# Autodesk Inventor assembly: buck-converter-din-rail-mount
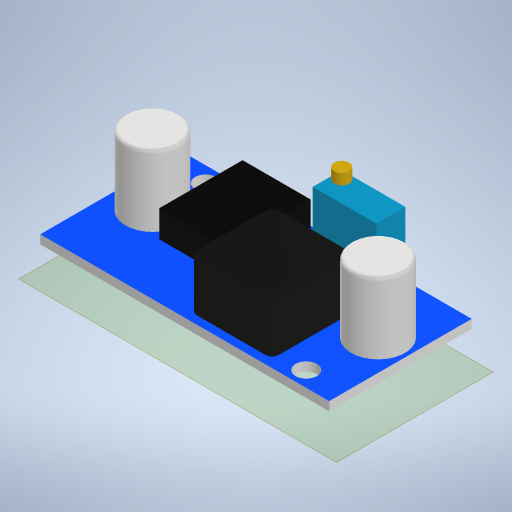
[picture p0: Inventor's stored thumbnail of the model, 512x512]
Saved by Autodesk Inventor 2023 (Build 270158030, 158C)
## iProperties
Created: 2024-03-29
Part Number: buck-converter-din-rail-mount
Document SubType Name: Assembly
Designer: Imogen Heard
Author: Imogen Heard
## iProperties of the stored document Power Buck Converter.ipt
Created: 2022-05-13
Part Number: Power Buck Converter
Material: Generic
Document SubType Name: Modeling
Designer: Imogen Heard
Density: 1 g/cm^3
Appearance: Default
Title: D:\Inventor\STEP FOR KICAD\Power Buck Converter.stp
Author: dech3
Sending System: Autodesk Inventor 2022
Preprocessor: ST-DEVELOPER v18.1
## Documents named in this file (3)
- **C:\Users\dheard\Documents\0004-inventor\Inventor_Projects\electronics-enclosure\buck-converter-din-rail-mount.iam*LocalDocs*xAaaaqqcaAaaaaaaaAaaaqi10Rg*Power Buck Converter.ipt
- C:\Users\dheard\Documents\0004-inventor\Inventor_Projects\electronics-enclosure\buck-converter-din-rail-mount.iam
- C:\Users\dheard\Documents\0004-inventor\Inventor_Projects\electronics-enclosure\Power Buck Converter.stp
## Components (1 placed, 1 different names)
1. Power Buck Converter:1 — Flush:1
## Relationships (1: Flush 1)
- Flush:1 (5 mm): Power Buck Converter:1
